# Autodesk Inventor assembly: SUBWashPiston
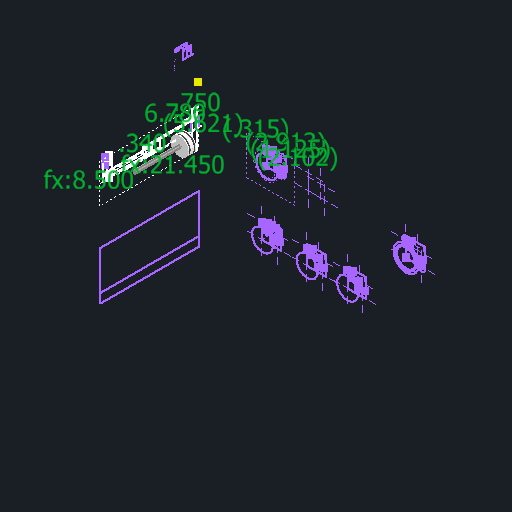
[picture p0: Inventor's stored thumbnail of the model, 512x512]
Saved by Autodesk Inventor 2024 (Build 280153000, 153)
## iProperties
Created: 2025-02-07
Part Number: SUBWashPiston
Document SubType Name: Assembly
Designer: Tommy Rohmann
Author: Tommy Rohmann
## Documents named in this file (5)
- C:\Users\Tommy Rohmann\OneDrive\Projects\Microgravity-Press-Washing-Machine\System Design and Documentation\Inventor Design Project\SUBWashPiston.iam
- C:\Users\Tommy Rohmann\OneDrive\Projects\Microgravity-Press-Washing-Machine\System Design and Documentation\Inventor Design Project\LAYOUT.ipt
- C:\Users\Tommy Rohmann\OneDrive\Projects\Microgravity-Press-Washing-Machine\System Design and Documentation\Inventor Design Project\WashPiston.ipt
- C:\Users\Tommy Rohmann\OneDrive\Projects\Microgravity-Press-Washing-Machine\System Design and Documentation\Inventor Design Project\DynamicPistonSeal.ipt
- C:\Users\Tommy Rohmann\OneDrive\Projects\Microgravity-Press-Washing-Machine\System Design and Documentation\Inventor Design Project\WashPistonRod.ipt
## Components (5 placed, 4 different names)
1. LAYOUT:1
2. WashPiston:1 — Mate:1, Mate:2, Mate:3, Mate:4, Mate:5, Mate:6
3. DynamicPistonSeal:1 — Mate:1, Mate:3
4. DynamicPistonSeal:2 — Mate:2, Mate:4
5. WashPistonRod:1 — Mate:5, Mate:6
## Relationships (8: Mate 6, Composite 2)
- [Composite]: LAYOUT:1 ↔ WashPiston:1
- Mate:1: WashPiston:1 ↔ DynamicPistonSeal:1
- Mate:2: WashPiston:1 ↔ DynamicPistonSeal:2
- Mate:3: WashPiston:1 ↔ DynamicPistonSeal:1
- Mate:4: WashPiston:1 ↔ DynamicPistonSeal:2
- [Composite]: LAYOUT:1 ↔ WashPistonRod:1
- Mate:5: WashPiston:1 ↔ WashPistonRod:1
- Mate:6: WashPiston:1 ↔ WashPistonRod:1
